# Autodesk Inventor assembly: Assembly1
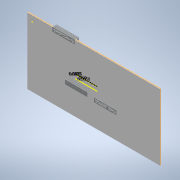
[picture p0: Inventor's stored thumbnail of the model, 180x180]
Saved by Autodesk Inventor 2020.2 (Build 242310000, 310)
## iProperties
Created: 2020-04-02
Part Number: Assembly1
Document SubType Name: Assembly
Designer: deli
Author: deli
## Documents named in this file (4)
- C:\Users\deli\OneDrive - Eastside Preparatory School\FTC\Chassi\Assembly1.iam
- C:\Users\deli\OneDrive - Eastside Preparatory School\FTC\Chassi\spoil board.ipt
- C:\Users\deli\OneDrive - Eastside Preparatory School\FTC\Chassi\Side Channel.ipt
- C:\Users\deli\OneDrive - Eastside Preparatory School\FTC\Chassi\metal jig.ipt
## Components (5 placed, 3 different names)
1. spoil board:1 — Mate:1
2. Side Channel:1
3. Side Channel:2
4. Side Channel:4
5. metal jig:1 — Mate:1
## Relationships (1: Mate 1)
- Mate:1: spoil board:1 ↔ metal jig:1
